# Autodesk Inventor assembly: Assembly1
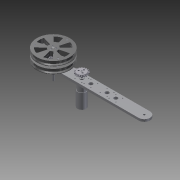
[picture p0: Inventor's stored thumbnail of the model, 180x180]
Saved by Autodesk Inventor 2011 (Build 150239000, 239)
## iProperties
Created: 2010-04-19
Part Number: Assembly1
Document SubType Name: Assembly
Designer: lucio
Author: lucio
## Documents named in this file (6)
- C:\Users\lucio\Documents\Inventor\caterpillar\Assembly1.iam
- C:\Users\lucio\Documents\Inventor\caterpillar\base side.ipt
- C:\Users\lucio\Documents\Inventor\caterpillar\mr85vel 2 etapas.ipt
- C:\Users\lucio\Documents\Inventor\caterpillar\back axle.ipt
- C:\Users\lucio\Documents\Inventor\caterpillar\back wheel.iam
- C:\Users\lucio\Documents\Inventor\caterpillar\sprocket.ipt
## Components (5 placed, 5 different names)
1. base side:1 — Insert:1, Mate:3, Mate:4
2. mr85vel 2 etapas:1 — Insert:1, Mate:5, Flush:1
3. back axle:1 — Mate:1, Mate:2, Mate:3
4. back wheel:1 [sub-assembly] — Mate:1, Mate:2, Mate:4
5. sprocket:1 — Mate:5, Flush:1
## Relationships (7: Mate 5, Insert 1, Flush 1)
- Mate:1: back axle:1 ↔ back wheel:1
- Insert:1: base side:1 ↔ mr85vel 2 etapas:1
- Mate:2: back axle:1 ↔ back wheel:1
- Mate:3: base side:1 ↔ back axle:1
- Mate:4 (5 mm): base side:1 ↔ back wheel:1
- Mate:5: mr85vel 2 etapas:1 ↔ sprocket:1
- Flush:1: mr85vel 2 etapas:1 ↔ sprocket:1
